# Autodesk Inventor assembly: full assembly draft
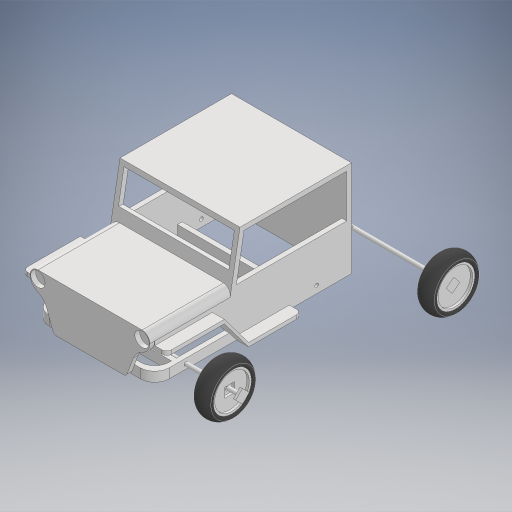
[picture p0: Inventor's stored thumbnail of the model, 512x512]
Saved by Autodesk Inventor 2024 (Build 280153000, 153)
## iProperties
Created: 2024-04-12
Part Number: full assembly draft
Document SubType Name: Assembly
Designer: Alex
Author: Alex
## Documents named in this file (5)
- C:\Shared\alex-bartella-schoolwork\4z03\final\final\full assembly draft.iam
- C:\Shared\alex-bartella-schoolwork\4z03\final\shell.ipt
- C:\Shared\alex-bartella-schoolwork\4z03\final\rear axle.ipt
- C:\Shared\alex-bartella-schoolwork\4z03\final\final\wheel.iam
- C:\Shared\alex-bartella-schoolwork\4z03\final\front axle.ipt
## Components (6 placed, 4 different names)
1. shell:1 — Mate:1, Mate:3, Mate:5, Mate:6, Mate:8
2. rear axle:1 — Mate:1, Mate:2, Mate:4, Mate:7
3. wheel:1 [sub-assembly] — Mate:2, Mate:3, Mate:4
4. wheel:2 [sub-assembly] — Mate:5, Mate:6, Mate:7
5. front axle:1 — Mate:8
6. wheel:3 [sub-assembly]
## Relationships (8: Mate 8)
- Mate:1: shell:1 ↔ rear axle:1
- Mate:2: rear axle:1 ↔ wheel:1
- Mate:3: shell:1 ↔ wheel:1
- Mate:4: rear axle:1 ↔ wheel:1
- Mate:5: shell:1 ↔ wheel:2
- Mate:6: shell:1 ↔ wheel:2
- Mate:7: rear axle:1 ↔ wheel:2
- Mate:8: shell:1 ↔ front axle:1
